# Autodesk Inventor assembly: Assembly
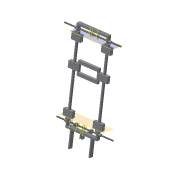
[picture p0: Inventor's stored thumbnail of the model, 180x180]
Saved by Autodesk Inventor 2018 (Build 220112000, 112)
## iProperties
Created: 2017-11-06
Part Number: Assembly
Document SubType Name: Assembly
Designer: David Cutting
Author: David Cutting
## Documents named in this file (10)
- C:\Users\davec\Documents\GitHub\Mousetrap\Assembly.iam
- C:\Users\davec\Documents\GitHub\Mousetrap\frontChassis_final.ipt
- C:\Users\davec\Documents\GitHub\Mousetrap\carbonFiberTube.ipt
- C:\Users\davec\Documents\GitHub\Mousetrap\clampCap.ipt
- C:\Users\davec\Documents\GitHub\Mousetrap\rearChassis_final.ipt
- C:\Users\davec\Documents\GitHub\Mousetrap\mousetrapHolder.ipt
- C:\Users\davec\Documents\GitHub\Mousetrap\535018\bearings.ipt
- C:\Users\davec\Documents\GitHub\Mousetrap\98873A200_MOISTURE-RESISTANT ACETAL THREADED ROD.ipt
- C:\Users\davec\Documents\GitHub\Mousetrap\nutSecurer.ipt
- C:\Users\davec\Documents\GitHub\Mousetrap\99223A029_ACETAL HEX NUT.ipt
## Components (27 placed, 9 different names)
1. frontChassis_final:1 — Mate:1, Mate:2, Mate:3, Mate:4, Angle:3, Flush:3, Angle:4, Flush:4, Mate:16, Mate:17, Mate:18, Mate:19, Mate:24, Mate:25, Mate:26, Mate:27
2. carbonFiberTube:1 — Mate:1, Mate:2, Mate:6, Mate:9, Mate:10, Mate:12, Mate:14
3. carbonFiberTube:2 — Mate:3, Mate:4, Mate:5, Mate:7, Mate:8, Mate:11, Mate:13, Mate:15
4. clampCap:1 — Mate:8, Angle:1, Flush:1
5. clampCap:2 — Mate:9, Angle:2, Flush:2
6. rearChassis_final:1 — Mate:5, Mate:6, Mate:7, Angle:1, Flush:1, Angle:2, Flush:2, Mate:20, Mate:21, Mate:22, Mate:23, Mate:31
7. clampCap:3 — Mate:10, Angle:3, Flush:3
8. clampCap:4 — Mate:11, Angle:4, Flush:4
9. mousetrapHolder:1 — Mate:12, Mate:13, Angle:5, Flush:5, Angle:6, Flush:6
10. clampCap:5 — Mate:15, Angle:6, Flush:6
11. clampCap:6 — Mate:14, Angle:5, Flush:5
12. bearings:1 — Mate:16, Mate:17, Mate:29, Mate:35
13. bearings:2 — Mate:26, Mate:27
14. bearings:3 — Mate:18, Mate:19, Mate:28, Mate:39
15. bearings:4 — Mate:20, Mate:21, Mate:33
16. bearings:5 — Mate:24, Mate:25
17. bearings:6 — Mate:22, Mate:23, Mate:30, Mate:37
18. 98873A200_MOISTURE-RESISTANT ACETAL THREADED ROD:1 — Mate:30, Mate:31, Mate:32, Mate:36, Mate:40, Mate:42
19. 98873A200_MOISTURE-RESISTANT ACETAL THREADED ROD:2 — Mate:28, Mate:29, Mate:34, Mate:38, Mate:44, Mate:46
20. nutSecurer:1 — Mate:34, Mate:35, Mate:47
21. nutSecurer:2 — Mate:36, Mate:37, Mate:41
22. nutSecurer:3 — Mate:32, Mate:33, Mate:43
23. nutSecurer:4 — Mate:38, Mate:39, Mate:45
24. 99223A029_ACETAL HEX NUT:1 — Mate:40, Mate:41
25. 99223A029_ACETAL HEX NUT:2 — Mate:42, Mate:43
26. 99223A029_ACETAL HEX NUT:3 — Mate:46, Mate:47
27. 99223A029_ACETAL HEX NUT:4 — Mate:44, Mate:45
## Relationships (59: Mate 47, Angle 6, Flush 6)
- Mate:1: frontChassis_final:1 ↔ carbonFiberTube:1
- Mate:2: frontChassis_final:1 ↔ carbonFiberTube:1
- Mate:3: frontChassis_final:1 ↔ carbonFiberTube:2
- Mate:4: frontChassis_final:1 ↔ carbonFiberTube:2
- Mate:5: carbonFiberTube:2 ↔ rearChassis_final:1
- Mate:6: carbonFiberTube:1 ↔ rearChassis_final:1
- Mate:7: carbonFiberTube:2 ↔ rearChassis_final:1
- Mate:8: carbonFiberTube:2 ↔ clampCap:1
- Angle:1 (0 deg): clampCap:1 ↔ rearChassis_final:1
- Flush:1: clampCap:1 ↔ rearChassis_final:1
- Mate:9: carbonFiberTube:1 ↔ clampCap:2
- Angle:2 (0 deg): clampCap:2 ↔ rearChassis_final:1
- Flush:2: clampCap:2 ↔ rearChassis_final:1
- Mate:10: carbonFiberTube:1 ↔ clampCap:3
- Angle:3 (0 deg): frontChassis_final:1 ↔ clampCap:3
- Flush:3: frontChassis_final:1 ↔ clampCap:3
- Mate:11: carbonFiberTube:2 ↔ clampCap:4
- Angle:4 (0 deg): frontChassis_final:1 ↔ clampCap:4
- Flush:4: frontChassis_final:1 ↔ clampCap:4
- Mate:12: carbonFiberTube:1 ↔ mousetrapHolder:1
- Mate:13: carbonFiberTube:2 ↔ mousetrapHolder:1
- Mate:14: carbonFiberTube:1 ↔ clampCap:6
- Angle:5 (0 deg): mousetrapHolder:1 ↔ clampCap:6
- Flush:5: mousetrapHolder:1 ↔ clampCap:6
- Mate:15: carbonFiberTube:2 ↔ clampCap:5
- Angle:6 (0 deg): mousetrapHolder:1 ↔ clampCap:5
- Flush:6: mousetrapHolder:1 ↔ clampCap:5
- Mate:16: frontChassis_final:1 ↔ bearings:1
- Mate:17: frontChassis_final:1 ↔ bearings:1
- Mate:18: frontChassis_final:1 ↔ bearings:3
- Mate:19: frontChassis_final:1 ↔ bearings:3
- Mate:20: rearChassis_final:1 ↔ bearings:4
- Mate:21: rearChassis_final:1 ↔ bearings:4
- Mate:22: rearChassis_final:1 ↔ bearings:6
- Mate:23: rearChassis_final:1 ↔ bearings:6
- Mate:24: frontChassis_final:1 ↔ bearings:5
- Mate:25: frontChassis_final:1 ↔ bearings:5
- Mate:26: frontChassis_final:1 ↔ bearings:2
- Mate:27: frontChassis_final:1 ↔ bearings:2
- Mate:28: bearings:3 ↔ 98873A200_MOISTURE-RESISTANT ACETAL THREADED ROD:2
- Mate:29: bearings:1 ↔ 98873A200_MOISTURE-RESISTANT ACETAL THREADED ROD:2
- Mate:30: bearings:6 ↔ 98873A200_MOISTURE-RESISTANT ACETAL THREADED ROD:1
- Mate:31: rearChassis_final:1 ↔ 98873A200_MOISTURE-RESISTANT ACETAL THREADED ROD:1
- Mate:32: 98873A200_MOISTURE-RESISTANT ACETAL THREADED ROD:1 ↔ nutSecurer:3
- Mate:33: bearings:4 ↔ nutSecurer:3
- Mate:34: 98873A200_MOISTURE-RESISTANT ACETAL THREADED ROD:2 ↔ nutSecurer:1
- Mate:35: bearings:1 ↔ nutSecurer:1
- Mate:36: 98873A200_MOISTURE-RESISTANT ACETAL THREADED ROD:1 ↔ nutSecurer:2
- Mate:37: bearings:6 ↔ nutSecurer:2
- Mate:38: 98873A200_MOISTURE-RESISTANT ACETAL THREADED ROD:2 ↔ nutSecurer:4
- Mate:39: bearings:3 ↔ nutSecurer:4
- Mate:40: 98873A200_MOISTURE-RESISTANT ACETAL THREADED ROD:1 ↔ 99223A029_ACETAL HEX NUT:1
- Mate:41: nutSecurer:2 ↔ 99223A029_ACETAL HEX NUT:1
- Mate:42: 98873A200_MOISTURE-RESISTANT ACETAL THREADED ROD:1 ↔ 99223A029_ACETAL HEX NUT:2
- Mate:43: nutSecurer:3 ↔ 99223A029_ACETAL HEX NUT:2
- Mate:44: 98873A200_MOISTURE-RESISTANT ACETAL THREADED ROD:2 ↔ 99223A029_ACETAL HEX NUT:4
- Mate:45: nutSecurer:4 ↔ 99223A029_ACETAL HEX NUT:4
- Mate:46: 98873A200_MOISTURE-RESISTANT ACETAL THREADED ROD:2 ↔ 99223A029_ACETAL HEX NUT:3
- Mate:47: nutSecurer:1 ↔ 99223A029_ACETAL HEX NUT:3
